# Autodesk Inventor assembly: rat_cap_EC_v12
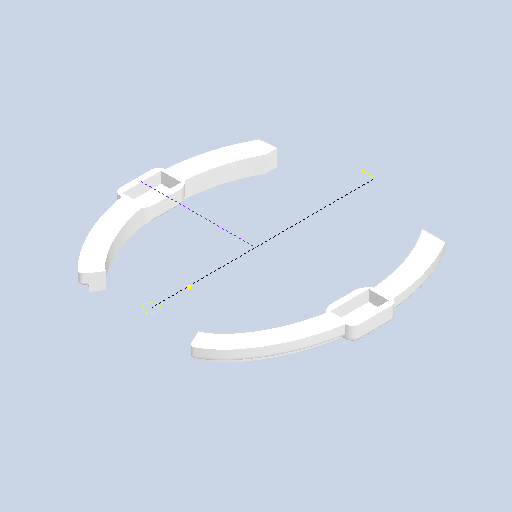
[picture p0: Inventor's stored thumbnail of the model, 512x512]
Saved by Autodesk Inventor 2025.4 (Build 294407000, 407)
## iProperties
Created: 2025-11-03
Part Number: rat_cap_EC_v12
Document SubType Name: Assembly
Designer: AdminForWorker
Title: rat_cap_EC_v12 v1
Author: AdminForWorker
## Documents named in this file (2)
- C:\Projects\Inventor\Misi cap system\Rat_cap\for Touchscreen setups\Rat_cap_with_lid\ipt_files\rat_cap_EC_v12.iam
- C:\Projects\Inventor\Misi cap system\Rat_cap\for Touchscreen setups\Rat_cap_with_lid\ipt_files\rat_cap_EC_v12 v0\rat_cap_walls_v8.iam
## Components (1 placed, 1 different names)
1. rat_cap_walls_v8:1 [sub-assembly]
## Named parameters: OuterWidth = 3 mm, OuterLength = 5.5 mm, InnerWidth = 2.5 mm, InnerLength = 5 mm
